# Autodesk Inventor assembly: mill_assembly
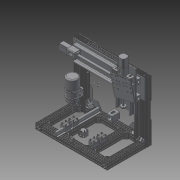
[picture p0: Inventor's stored thumbnail of the model, 180x180]
Saved by Autodesk Inventor 2014 (Build 180170000, 170)
## iProperties
Created: 2014-08-08
Part Number: mill_assembly
Document SubType Name: Assembly
Designer: Matthew
Author: Matthew
## Documents named in this file (43)
- C:\Users\matmell\Documents\GitHub\cncmill\mill_assembly.iam
- C:\Users\matmell\Documents\GitHub\cncmill\8020\2020.ipt
- C:\Users\matmell\Documents\GitHub\cncmill\8020\2020_18in.ipt
- C:\Users\matmell\Documents\GitHub\cncmill\8020\gusset_4138.ipt
- C:\Users\matmell\Documents\GitHub\cncmill\8020\gusset_4134.ipt
- C:\Users\matmell\Documents\GitHub\cncmill\mic6_plate.ipt
- C:\Users\matmell\Documents\GitHub\cncmill\1605\1605_400mm.ipt
- C:\Users\matmell\Documents\GitHub\cncmill\1605\1605_ballnut.ipt
- C:\Users\matmell\Documents\GitHub\cncmill\nema23_motor_mount.ipt
- C:\Users\matmell\Documents\GitHub\cncmill\6.35x10mm_coupler.ipt
- C:\Users\matmell\Documents\GitHub\cncmill\sbr\sbr20\sbr20_400mm.ipt
- C:\Users\matmell\Documents\GitHub\cncmill\HD16.ipt
- C:\Users\matmell\Documents\GitHub\cncmill\nema23_HS8630.ipt
- C:\Users\matmell\Documents\GitHub\cncmill\z-axis_mount_plate.ipt
- C:\Users\matmell\Documents\GitHub\cncmill\y-axis_mount_plate.ipt
- C:\Users\matmell\Documents\GitHub\cncmill\router_plate.ipt
- C:\Users\matmell\Documents\GitHub\cncmill\router_mount.ipt
- C:\Users\matmell\Documents\GitHub\cncmill\1617evs.ipt
- C:\Users\matmell\Documents\GitHub\cncmill\ff12_mount.ipt
- C:\Users\matmell\Documents\GitHub\cncmill\ff12.ipt
- C:\Users\matmell\Documents\GitHub\cncmill\sbr\sbr20\sbr20_500mm.ipt
- C:\Users\matmell\Documents\GitHub\cncmill\1605\1605_500mm.ipt
- C:\Users\matmell\Documents\GitHub\cncmill\sbr\sbr20\sbr20_300mm.ipt
- C:\Users\matmell\Documents\GitHub\cncmill\8020\2040_top_bar.ipt
- C:\Users\matmell\Documents\GitHub\cncmill\8020\2040_uprights.ipt
- C:\Users\matmell\Documents\GitHub\cncmill\8020\2020_rear.ipt
- C:\Users\matmell\Documents\GitHub\cncmill\8020\2020_front.ipt
- C:\Users\matmell\Documents\GitHub\cncmill\1605\1605_300mm.ipt
- C:\Users\matmell\Documents\GitHub\cncmill\versaframe\versaframe_30in.ipt
- C:\Users\matmell\Documents\GitHub\cncmill\versaframe\versaframe_35in.ipt
- C:\Users\matmell\Documents\GitHub\cncmill\versaframe\versaframe_7.5n.ipt
- C:\Users\matmell\Documents\GitHub\cncmill\8020\2040-2040_left.iam
- C:\Users\matmell\Documents\GitHub\cncmill\8020\2040-2040_right.iam
- C:\Users\matmell\Documents\GitHub\cncmill\8020\2020-2040_right.iam
- C:\Users\matmell\Documents\GitHub\cncmill\8020\2020-2040_left.iam
- C:\Users\matmell\Documents\GitHub\cncmill\fk12.ipt
- C:\Users\matmell\Documents\GitHub\cncmill\sbr\sbr20\sbr20uu.ipt
- C:\Users\matmell\Documents\GitHub\cncmill\m6x1.ipt
- C:\Users\matmell\Documents\GitHub\cncmill\m5x0.8.ipt
- C:\Users\matmell\Documents\GitHub\cncmill\8020\SHCS bolt.ipt
- C:\Users\matmell\Documents\GitHub\cncmill\8020\0.5in_tnut.iam
- C:\Users\matmell\Documents\GitHub\cncmill\Metric socket button head, Class 12.9 steel black oil finish, 5mm x.ipt
- C:\Users\matmell\Documents\GitHub\cncmill\Metric socket button head, Class 12.9 steel black oil finish, 6mm x 1.ipt
## Components (124 placed, 42 different names)
1. 2020_18in:1 — Mate:31, Mate:32, Mate:38, Mate:47, Mate:48, Flush:161, Flush:168, Mate:253
2. 2020_18in:2 — Mate:28, Mate:29, Mate:34, Mate:241, Flush:163, Mate:242, Flush:164, Mate:255, Flush:171, Flush:172, Mate:394
3. gusset_4138:1 — Mate:260, Mate:261, Flush:175
4. gusset_4138:2 — Mate:258, Mate:259, Mate:262, Flush:175
5. gusset_4134:1 — Mate:28, Mate:29, Mate:275
6. gusset_4134:2 — Mate:31, Mate:32, Mate:276, Insert:58, Insert:60, Insert:61, Insert:62
7. gusset_4134:3 — Mate:34, Flush:61, Flush:147, Mate:278
8. gusset_4134:4 — Mate:38, Flush:62, Flush:153, Mate:279
9. gusset_4134:6 — Mate:47, Mate:48, Flush:61, Flush:62, Mate:269, Flush:401, Flush:402, Flush:403
10. mic6_plate:1 — Insert:17, Insert:18, Insert:19, Insert:20, Insert:21, Insert:22, Insert:23, Insert:24, Insert:25, Insert:26, Insert:27, Insert:28, Insert:29, Insert:30, Insert:31, Insert:32, Insert:33, Insert:34, Insert:35, Insert:36, Flush:395, Mate:397
11. 1605_400mm:1 — Mate:108, Insert:2, Insert:16, Mate:404, Flush:408
12. 1605_ballnut:1 — Mate:108, Mate:133, Mate:134, Mate:408
13. nema23_motor_mount:1 — Mate:136, Mate:254, Flush:192, Flush:193, Mate:317, Flush:329, Flush:330, Flush:407
14. nema23_motor_mount:2 — Mate:154, Flush:321, Flush:322, Mate:316, Flush:327, Flush:328, Mate:364, Flush:376
15. 1605_ballnut:6 — Mate:158, Mate:159, Mate:282
16. 6.35x10mm_coupler:1 — Insert:4, Insert:14
17. sbr20_400mm:1 — Flush:136, Mate:247, Flush:191, Mate:318
18. sbr20_400mm:2 — Flush:136, Mate:248, Flush:190, Mate:328
19. HD16:1 — Mate:133, Mate:134, Mate:326, Mate:329, Mate:395, Mate:408
20. nema23_HS8630:1 — Mate:136, Flush:192, Flush:193
21. 6.35x10mm_coupler:2 — Insert:2
22. z-axis_mount_plate:1 — Flush:370, Flush:371, Flush:372, Flush:373, Mate:362, Mate:363, Flush:375, Mate:364, Flush:376, Flush:390, Mate:400, Angle:2
23. nema23_HS8630:2 — Mate:154, Insert:4, Flush:321, Flush:322
24. HD16:6 — Mate:158, Mate:159, Mate:210, Mate:211, Flush:390, Mate:405, Mate:406
25. y-axis_mount_plate:1 — Mate:177, Mate:199, Mate:200, Flush:135, Mate:206, Flush:137, Flush:184, Mate:267, Flush:396
26. nema23_motor_mount:4 — Mate:177, Flush:137, Flush:323, Flush:324, Mate:315, Flush:325, Flush:326
27. 6.35x10mm_coupler:3
28. nema23_HS8630:3 — Flush:323, Flush:324
29. 1605_ballnut:7 — Mate:240
30. HD16:7 — Mate:203, Mate:205, Mate:348
31. router_mount:1 — Insert:7
32. 1617evs:1 — Insert:7
33. ff12:1 — Mate:404, Flush:408, Angle:1
34. sbr20_500mm:1 — Flush:133, Mate:200, Mate:203, Flush:135, Mate:346, Flush:371, Mate:382
35. sbr20_500mm:2 — Flush:133, Mate:199, Mate:205, Mate:347
36. 1605_500mm:1 — Insert:11, Mate:240, Insert:15
37. ff12:2 — Insert:11, Insert:12
38. ff12_mount:2 — Insert:12, Mate:206
39. sbr20_300mm:1 — Flush:138, Mate:210, Flush:372, Mate:363, Flush:374, Flush:375, Mate:371
40. sbr20_300mm:2 — Flush:138, Mate:211, Flush:373, Mate:362, Flush:374, Mate:377
41. 2020:1 — Mate:223, Mate:230, Mate:233, Mate:248, Flush:169, Flush:190, Mate:389, Mate:398
42. 2020:2 — Mate:222, Mate:224, Mate:226, Mate:247, Flush:170, Flush:191, Mate:391, Mate:403
43. gusset_4134:8 — Mate:222, Flush:147, Mate:277
44. gusset_4134:9 — Mate:223, Flush:149, Flush:150, Flush:151, Mate:280, Flush:401
45. gusset_4134:11 — Mate:224, Flush:149, Mate:268
46. gusset_4134:12 — Mate:230, Flush:151, Mate:390
47. gusset_4134:13 — Mate:226, Flush:150, Mate:281
48. gusset_4134:14 — Flush:153, Mate:233
49. 2040_top_bar:1 — Mate:257, Flush:173, Flush:174, Mate:258, Mate:261, Flush:184, Mate:267, Flush:313, Flush:315
50. 2040_uprights:1 — Flush:161, Mate:241, Flush:167, Mate:252, Flush:168, Mate:253, Mate:257, Flush:173, Flush:174, Mate:259, Mate:262, Mate:269, Mate:276, Mate:311, Flush:314, Mate:314, Flush:319, Flush:320, Flush:396, Flush:398, Mate:385, Flush:400, Mate:395
51. 2040_uprights:2 — Flush:163, Mate:242, Flush:164, Mate:249, Flush:165, Flush:166, Mate:260, Mate:275, Flush:208, Mate:312, Flush:316, Mate:313, Flush:317, Flush:318, Mate:386, Flush:399, Flush:404, Mate:393
52. 2020_rear:1 — Mate:249, Flush:165, Flush:166, Flush:167, Mate:252, Flush:169, Flush:170, Mate:254, Mate:268, Mate:280, Flush:221, Mate:384, Mate:387, Mate:388, Mate:392, Flush:407
53. 2020_front:1 — Mate:255, Flush:171, Flush:172, Mate:277, Mate:278, Mate:279, Mate:281, Mate:390, Mate:398, Mate:403, Angle:1
54. 1605_300mm:1 — Insert:14, Mate:282, Insert:69
55. versaframe_30in:1 — Flush:200, Flush:201, Mate:294, Flush:202, Flush:203, Mate:295, Flush:205, Flush:206, Flush:228, Flush:230
56. versaframe_30in:2 — Flush:200, Flush:201, Flush:204, Flush:221
57. versaframe_35in:1 — Mate:294, Flush:202, Flush:203, Flush:204, Flush:208, Flush:213, Mate:303, Flush:229
58. versaframe_35in:2 — Mate:295, Flush:205, Flush:206, Mate:297, Flush:209, Flush:210, Mate:304, Flush:231
59. versaframe_30in:3 — Mate:297, Flush:209, Flush:210, Flush:211, Flush:212, Flush:232, Flush:233, Mate:305
60. versaframe_30in:4 — Flush:211, Flush:212, Flush:213, Flush:220, Flush:308, Flush:235, Flush:309
61. versaframe_7.5n:1 — Flush:308, Flush:235, Flush:309, Flush:310, Flush:311, Mate:307, Mate:308
62. versaframe_7.5n:2 — Flush:232, Flush:233, Mate:305, Mate:306, Flush:234, Mate:309, Mate:310, Flush:312
63. versaframe_30in:5 — Flush:220, Flush:222, Mate:306, Flush:234, Flush:310
64. versaframe_30in:6 — Flush:222, Flush:311, Mate:307, Mate:308
65. versaframe_7.5n:3 — Mate:303, Flush:228, Flush:229
66. versaframe_7.5n:4 — Mate:304, Flush:230, Flush:231
67. versaframe_30in:7
68. versaframe_30in:8 — Mate:309, Mate:310, Flush:312
69. 2040-2040_left:1 [sub-assembly] — Mate:311, Flush:313, Flush:314
70. 2040-2040_right:1 [sub-assembly] — Mate:312, Flush:315, Flush:316
71. 2020-2040_right:1 [sub-assembly] — Mate:313, Flush:317, Flush:318
72. 2020-2040_left:1 [sub-assembly] — Mate:314, Flush:319, Flush:320
73. fk12:1 — Insert:15, Mate:315, Flush:325, Flush:326, Mate:382
74. fk12:2 — Mate:316, Flush:327, Flush:328
75. fk12:3 — Mate:317, Flush:329, Flush:330, Insert:16
76. sbr20uu:1 — Flush:332, Mate:319, Flush:333, Mate:396, Mate:397
77. sbr20uu:2 — Mate:318, Flush:332, Mate:319, Flush:333, Mate:326, Flush:395, Flush:406
78. sbr20uu:3 — Flush:344, Mate:327, Flush:345, Mate:328, Mate:329, Flush:406
79. sbr20uu:13 — Flush:344, Mate:327, Flush:345
80. m6x1:1 — Insert:24
81. m6x1:2 — Insert:21
82. m6x1:3 — Insert:17
83. m6x1:4 — Insert:20
84. m6x1:5 — Insert:18
85. m6x1:6 — Insert:19
86. m6x1:7 — Insert:22
87. m6x1:8 — Insert:23
88. m6x1:9 — Insert:28
89. m6x1:10 — Insert:27
90. m6x1:11 — Insert:32, Mate:396
91. m6x1:12 — Insert:26
92. m6x1:13 — Insert:29
93. m6x1:14 — Insert:30
94. m6x1:15 — Insert:25
95. m6x1:16 — Insert:31
96. m5x0.8:1 — Insert:36
97. m5x0.8:2 — Insert:34
98. m5x0.8:3 — Insert:33
99. m5x0.8:4 — Insert:35
100. sbr20uu:14 — Mate:347, Flush:362, Mate:348, Flush:370
101. sbr20uu:15
102. sbr20uu:18 — Mate:346, Flush:362
103. sbr20uu:19 — Mate:400
104. sbr20uu:22 — Mate:371
105. sbr20uu:23 — Flush:387, Mate:407
106. sbr20uu:24
107. sbr20uu:25 — Mate:377, Flush:387
108. gusset_4138:5 — Mate:384, Flush:398, Mate:385
109. gusset_4138:6 — Mate:386, Flush:399, Mate:387
110. gusset_4134:15 — Mate:388, Mate:389, Flush:400, Flush:402
111. gusset_4134:16 — Mate:391, Flush:403, Flush:404, Mate:392, Flush:405
112. gusset_4134:17 — Mate:393, Mate:394, Flush:405
113. SHCS bolt:2 — Insert:58
114. 0.5in_tnut:2 [sub-assembly] — Insert:60
115. 0.5in_tnut:3 [sub-assembly] — Insert:61
116. SHCS bolt:3 — Insert:62
117. Metric socket button head, Class 12.9 steel black oil finish, 5mm x:1
118. Metric socket button head, Class 12.9 steel black oil finish, 5mm x:2 — Mate:405
119. Metric socket button head, Class 12.9 steel black oil finish, 5mm x:3
120. Metric socket button head, Class 12.9 steel black oil finish, 5mm x:4
121. Metric socket button head, Class 12.9 steel black oil finish, 6mm x 1:1
122. Metric socket button head, Class 12.9 steel black oil finish, 6mm x 1:2
123. ff12:3 — Insert:69, Angle:2
124. router_plate:1 — Mate:406, Mate:407
## Relationships (267: Mate 118, Flush 113, Insert 34, Angle 2)
- Mate:28: 2020_18in:2 ↔ gusset_4134:1
- Mate:29: 2020_18in:2 ↔ gusset_4134:1
- Mate:31: 2020_18in:1 ↔ gusset_4134:2
- Mate:32: 2020_18in:1 ↔ gusset_4134:2
- Mate:34: 2020_18in:2 ↔ gusset_4134:3
- Mate:38: 2020_18in:1 ↔ gusset_4134:4
- Mate:47: 2020_18in:1 ↔ gusset_4134:6
- Mate:48: 2020_18in:1 ↔ gusset_4134:6
- Mate:108: 1605_400mm:1 ↔ 1605_ballnut:1
- Flush:61: gusset_4134:3 ↔ gusset_4134:6
- Flush:62: gusset_4134:4 ↔ gusset_4134:6
- Mate:133: 1605_ballnut:1 ↔ HD16:1
- Mate:134: 1605_ballnut:1 ↔ HD16:1
- Insert:2 (-12.5 mm): 1605_400mm:1 ↔ 6.35x10mm_coupler:2
- Mate:136: nema23_motor_mount:1 ↔ nema23_HS8630:1
- Mate:154: nema23_motor_mount:2 ↔ nema23_HS8630:2
- Insert:4 (-7 mm): 6.35x10mm_coupler:1 ↔ nema23_HS8630:2
- Mate:158: 1605_ballnut:6 ↔ HD16:6
- Mate:159: 1605_ballnut:6 ↔ HD16:6
- [Mate]: nema23_motor_mount:4 ↔ nema23_HS8630:3
- [Insert] (-7 mm): 6.35x10mm_coupler:3 ↔ nema23_HS8630:3
- [Mate]: 1605_ballnut:7 ↔ HD16:7
- [Mate]: 1605_ballnut:7 ↔ HD16:7
- Mate:177: y-axis_mount_plate:1 ↔ nema23_motor_mount:4
- Insert:7: router_mount:1 ↔ 1617evs:1
- Flush:133: sbr20_500mm:1 ↔ sbr20_500mm:2
- Mate:199: y-axis_mount_plate:1 ↔ sbr20_500mm:2
- Mate:200: y-axis_mount_plate:1 ↔ sbr20_500mm:1
- Mate:203 (19.9 mm): HD16:7 ↔ sbr20_500mm:1
- Mate:205 (19.9 mm): HD16:7 ↔ sbr20_500mm:2
- Flush:135: y-axis_mount_plate:1 ↔ sbr20_500mm:1
- Flush:136: sbr20_400mm:1 ↔ sbr20_400mm:2
- Insert:11: 1605_500mm:1 ↔ ff12:2
- Insert:12: ff12:2 ↔ ff12_mount:2
- Mate:206: y-axis_mount_plate:1 ↔ ff12_mount:2
- Flush:137: y-axis_mount_plate:1 ↔ nema23_motor_mount:4
- Flush:138: sbr20_300mm:1 ↔ sbr20_300mm:2
- Mate:210 (11 mm): HD16:6 ↔ sbr20_300mm:1
- Mate:211 (11 mm): HD16:6 ↔ sbr20_300mm:2
- Mate:222: 2020:2 ↔ gusset_4134:8
- Flush:147: gusset_4134:3 ↔ gusset_4134:8
- Mate:223: 2020:1 ↔ gusset_4134:9
- Mate:224: 2020:2 ↔ gusset_4134:11
- Mate:226: 2020:2 ↔ gusset_4134:13
- Flush:149: gusset_4134:9 ↔ gusset_4134:11
- Mate:230: 2020:1 ↔ gusset_4134:12
- Flush:150: gusset_4134:9 ↔ gusset_4134:13
- Flush:151: gusset_4134:9 ↔ gusset_4134:12
- Flush:153: gusset_4134:4 ↔ gusset_4134:14
- Mate:233: 2020:1 ↔ gusset_4134:14
- Mate:240: 1605_ballnut:7 ↔ 1605_500mm:1
- Flush:161: 2020_18in:1 ↔ 2040_uprights:1
- Mate:241: 2020_18in:2 ↔ 2040_uprights:1
- Flush:163: 2020_18in:2 ↔ 2040_uprights:2
- Mate:242: 2020_18in:2 ↔ 2040_uprights:2
- Flush:164: 2020_18in:2 ↔ 2040_uprights:2
- Mate:247: sbr20_400mm:1 ↔ 2020:2
- Mate:248: sbr20_400mm:2 ↔ 2020:1
- Mate:249: 2040_uprights:2 ↔ 2020_rear:1
- Flush:165: 2040_uprights:2 ↔ 2020_rear:1
- Flush:166: 2040_uprights:2 ↔ 2020_rear:1
- Flush:167: 2040_uprights:1 ↔ 2020_rear:1
- Mate:252: 2040_uprights:1 ↔ 2020_rear:1
- Flush:168: 2020_18in:1 ↔ 2040_uprights:1
- Mate:253: 2020_18in:1 ↔ 2040_uprights:1
- Flush:169: 2020:1 ↔ 2020_rear:1
- Flush:170: 2020:2 ↔ 2020_rear:1
- Mate:254: nema23_motor_mount:1 ↔ 2020_rear:1
- Mate:255: 2020_18in:2 ↔ 2020_front:1
- Flush:171: 2020_18in:2 ↔ 2020_front:1
- Flush:172: 2020_18in:2 ↔ 2020_front:1
- Mate:257: 2040_top_bar:1 ↔ 2040_uprights:1
- Flush:173: 2040_top_bar:1 ↔ 2040_uprights:1
- Flush:174: 2040_top_bar:1 ↔ 2040_uprights:1
- Mate:258: gusset_4138:2 ↔ 2040_top_bar:1
- Mate:259: gusset_4138:2 ↔ 2040_uprights:1
- Mate:260: gusset_4138:1 ↔ 2040_uprights:2
- Mate:261: gusset_4138:1 ↔ 2040_top_bar:1
- Mate:262: gusset_4138:2 ↔ 2040_uprights:1
- Flush:175: gusset_4138:1 ↔ gusset_4138:2
- Flush:184: y-axis_mount_plate:1 ↔ 2040_top_bar:1
- Mate:267: y-axis_mount_plate:1 ↔ 2040_top_bar:1
- Mate:268: gusset_4134:11 ↔ 2020_rear:1
- Mate:269: gusset_4134:6 ↔ 2040_uprights:1
- Flush:190: sbr20_400mm:2 ↔ 2020:1
- Flush:191: sbr20_400mm:1 ↔ 2020:2
- Mate:275: gusset_4134:1 ↔ 2040_uprights:2
- Mate:276: gusset_4134:2 ↔ 2040_uprights:1
- Mate:277: gusset_4134:8 ↔ 2020_front:1
- Mate:278: gusset_4134:3 ↔ 2020_front:1
- Mate:279: gusset_4134:4 ↔ 2020_front:1
- Mate:280: gusset_4134:9 ↔ 2020_rear:1
- Mate:281: gusset_4134:13 ↔ 2020_front:1
- Insert:14 (-12.5 mm): 6.35x10mm_coupler:1 ↔ 1605_300mm:1
- Mate:282: 1605_ballnut:6 ↔ 1605_300mm:1
- Flush:192 (-0.889 mm): nema23_motor_mount:1 ↔ nema23_HS8630:1
- Flush:193: nema23_motor_mount:1 ↔ nema23_HS8630:1
- Flush:200: versaframe_30in:1 ↔ versaframe_30in:2
- Flush:201: versaframe_30in:1 ↔ versaframe_30in:2
- Mate:294: versaframe_30in:1 ↔ versaframe_35in:1
- Flush:202: versaframe_30in:1 ↔ versaframe_35in:1
- Flush:203: versaframe_30in:1 ↔ versaframe_35in:1
- Flush:204: versaframe_30in:2 ↔ versaframe_35in:1
- Mate:295: versaframe_30in:1 ↔ versaframe_35in:2
- Flush:205: versaframe_30in:1 ↔ versaframe_35in:2
- Flush:206: versaframe_30in:1 ↔ versaframe_35in:2
- Flush:208: 2040_uprights:2 ↔ versaframe_35in:1
- Mate:297: versaframe_35in:2 ↔ versaframe_30in:3
- Flush:209: versaframe_35in:2 ↔ versaframe_30in:3
- Flush:210: versaframe_35in:2 ↔ versaframe_30in:3
- Flush:211: versaframe_30in:3 ↔ versaframe_30in:4
- Flush:212: versaframe_30in:3 ↔ versaframe_30in:4
- Flush:213: versaframe_35in:1 ↔ versaframe_30in:4
- Flush:220: versaframe_30in:4 ↔ versaframe_30in:5
- Flush:221: 2020_rear:1 ↔ versaframe_30in:2
- Flush:222: versaframe_30in:5 ↔ versaframe_30in:6
- Mate:303: versaframe_35in:1 ↔ versaframe_7.5n:3
- Flush:228: versaframe_30in:1 ↔ versaframe_7.5n:3
- Flush:229: versaframe_35in:1 ↔ versaframe_7.5n:3
- Mate:304: versaframe_35in:2 ↔ versaframe_7.5n:4
- Flush:230: versaframe_30in:1 ↔ versaframe_7.5n:4
- Flush:231: versaframe_35in:2 ↔ versaframe_7.5n:4
- Flush:232: versaframe_30in:3 ↔ versaframe_7.5n:2
- Flush:233: versaframe_30in:3 ↔ versaframe_7.5n:2
- Mate:305: versaframe_30in:3 ↔ versaframe_7.5n:2
- Mate:306: versaframe_7.5n:2 ↔ versaframe_30in:5
- Flush:234: versaframe_7.5n:2 ↔ versaframe_30in:5
- Flush:308: versaframe_30in:4 ↔ versaframe_7.5n:1
- Flush:235: versaframe_30in:4 ↔ versaframe_7.5n:1
- Flush:309: versaframe_30in:4 ↔ versaframe_7.5n:1
- Flush:310: versaframe_7.5n:1 ↔ versaframe_30in:5
- Flush:311: versaframe_7.5n:1 ↔ versaframe_30in:6
- Mate:307: versaframe_7.5n:1 ↔ versaframe_30in:6
- Mate:308: versaframe_7.5n:1 ↔ versaframe_30in:6
- Mate:309: versaframe_7.5n:2 ↔ versaframe_30in:8
- Mate:310: versaframe_7.5n:2 ↔ versaframe_30in:8
- Flush:312: versaframe_7.5n:2 ↔ versaframe_30in:8
- Mate:311: 2040_uprights:1 ↔ 2040-2040_left:1
- Flush:313: 2040_top_bar:1 ↔ 2040-2040_left:1
- Flush:314: 2040_uprights:1 ↔ 2040-2040_left:1
- Mate:312: 2040_uprights:2 ↔ 2040-2040_right:1
- Flush:315: 2040_top_bar:1 ↔ 2040-2040_right:1
- Flush:316: 2040_uprights:2 ↔ 2040-2040_right:1
- Mate:313: 2040_uprights:2 ↔ 2020-2040_right:1
- Flush:317: 2040_uprights:2 ↔ 2020-2040_right:1
- Flush:318: 2040_uprights:2 ↔ 2020-2040_right:1
- Mate:314: 2040_uprights:1 ↔ 2020-2040_left:1
- Flush:319: 2040_uprights:1 ↔ 2020-2040_left:1
- Flush:320: 2040_uprights:1 ↔ 2020-2040_left:1
- Flush:321 (-0.889 mm): nema23_motor_mount:2 ↔ nema23_HS8630:2
- Flush:322 (0.889 mm): nema23_motor_mount:2 ↔ nema23_HS8630:2
- Flush:323 (-0.889 mm): nema23_motor_mount:4 ↔ nema23_HS8630:3
- Flush:324: nema23_motor_mount:4 ↔ nema23_HS8630:3
- Insert:15: 1605_500mm:1 ↔ fk12:1
- Mate:315: nema23_motor_mount:4 ↔ fk12:1
- Flush:325 (6.1305 mm): nema23_motor_mount:4 ↔ fk12:1
- Flush:326 (6.1305 mm): nema23_motor_mount:4 ↔ fk12:1
- Mate:316: nema23_motor_mount:2 ↔ fk12:2
- Flush:327 (-6.1305 mm): nema23_motor_mount:2 ↔ fk12:2
- Flush:328 (6.1305 mm): nema23_motor_mount:2 ↔ fk12:2
- Mate:317: nema23_motor_mount:1 ↔ fk12:3
- Flush:329 (6.1305 mm): nema23_motor_mount:1 ↔ fk12:3
- Flush:330 (6.1305 mm): nema23_motor_mount:1 ↔ fk12:3
- Insert:16: 1605_400mm:1 ↔ fk12:3
- Mate:318: sbr20_400mm:1 ↔ sbr20uu:2
- Flush:332: sbr20uu:1 ↔ sbr20uu:2
- Mate:319 (20 mm): sbr20uu:1 ↔ sbr20uu:2
- Flush:333: sbr20uu:1 ↔ sbr20uu:2
- Mate:326 (-7.5 mm): HD16:1 ↔ sbr20uu:2
- Flush:344: sbr20uu:3 ↔ sbr20uu:13
- Mate:327 (20 mm): sbr20uu:3 ↔ sbr20uu:13
- Flush:345: sbr20uu:3 ↔ sbr20uu:13
- Mate:328: sbr20_400mm:2 ↔ sbr20uu:3
- Mate:329 (-7.5 mm): HD16:1 ↔ sbr20uu:3
- Insert:17: mic6_plate:1 ↔ m6x1:3
- Insert:18: mic6_plate:1 ↔ m6x1:5
- Insert:19: mic6_plate:1 ↔ m6x1:6
- Insert:20: mic6_plate:1 ↔ m6x1:4
- Insert:21: mic6_plate:1 ↔ m6x1:2
- Insert:22: mic6_plate:1 ↔ m6x1:7
- Insert:23: mic6_plate:1 ↔ m6x1:8
- Insert:24: mic6_plate:1 ↔ m6x1:1
- Insert:25: mic6_plate:1 ↔ m6x1:15
- Insert:26: mic6_plate:1 ↔ m6x1:12
- Insert:27: mic6_plate:1 ↔ m6x1:10
- Insert:28: mic6_plate:1 ↔ m6x1:9
- Insert:29: mic6_plate:1 ↔ m6x1:13
- Insert:30: mic6_plate:1 ↔ m6x1:14
- Insert:31: mic6_plate:1 ↔ m6x1:16
- Insert:32: mic6_plate:1 ↔ m6x1:11
- Insert:33: mic6_plate:1 ↔ m5x0.8:3
- Insert:34: mic6_plate:1 ↔ m5x0.8:2
- Insert:35: mic6_plate:1 ↔ m5x0.8:4
- Insert:36: mic6_plate:1 ↔ m5x0.8:1
- [Flush]: sbr20uu:14 ↔ sbr20uu:15
- [Mate] (60 mm): sbr20uu:14 ↔ sbr20uu:15
- [Flush]: sbr20uu:14 ↔ sbr20uu:15
- [Flush]: sbr20uu:18 ↔ sbr20uu:19
- [Mate] (70 mm): sbr20uu:18 ↔ sbr20uu:19
- [Flush]: sbr20uu:18 ↔ sbr20uu:19
- Mate:346: sbr20_500mm:1 ↔ sbr20uu:18
- Mate:347: sbr20_500mm:2 ↔ sbr20uu:14
- Flush:362: sbr20uu:14 ↔ sbr20uu:18
- Mate:348 (12.5 mm): HD16:7 ↔ sbr20uu:14
- Flush:370: z-axis_mount_plate:1 ↔ sbr20uu:14
- Flush:371 (-91.0209 mm): z-axis_mount_plate:1 ↔ sbr20_500mm:1
- Flush:372: z-axis_mount_plate:1 ↔ sbr20_300mm:1
- Flush:373: z-axis_mount_plate:1 ↔ sbr20_300mm:2
- Mate:362: z-axis_mount_plate:1 ↔ sbr20_300mm:2
- Mate:363: z-axis_mount_plate:1 ↔ sbr20_300mm:1
- Flush:374: sbr20_300mm:1 ↔ sbr20_300mm:2
- Flush:375: z-axis_mount_plate:1 ↔ sbr20_300mm:1
- Mate:364: nema23_motor_mount:2 ↔ z-axis_mount_plate:1
- Flush:376: nema23_motor_mount:2 ↔ z-axis_mount_plate:1
- [Flush]: sbr20uu:22 ↔ sbr20uu:23
- [Mate] (10 mm): sbr20uu:22 ↔ sbr20uu:23
- [Flush]: sbr20uu:22 ↔ sbr20uu:23
- Mate:371: sbr20_300mm:1 ↔ sbr20uu:22
- [Flush]: sbr20uu:24 ↔ sbr20uu:25
- [Mate] (10 mm): sbr20uu:24 ↔ sbr20uu:25
- [Flush]: sbr20uu:24 ↔ sbr20uu:25
- Mate:377: sbr20_300mm:2 ↔ sbr20uu:25
- Flush:387: sbr20uu:23 ↔ sbr20uu:25
- Flush:390 (61 mm): z-axis_mount_plate:1 ↔ HD16:6
- Mate:382 (-40 mm): sbr20_500mm:1 ↔ fk12:1
- Flush:395 (-92.4 mm): mic6_plate:1 ↔ sbr20uu:2
- Flush:396: y-axis_mount_plate:1 ↔ 2040_uprights:1
- Mate:384: 2020_rear:1 ↔ gusset_4138:5
- Flush:398: 2040_uprights:1 ↔ gusset_4138:5
- Mate:385: 2040_uprights:1 ↔ gusset_4138:5
- Mate:386: 2040_uprights:2 ↔ gusset_4138:6
- Flush:399: 2040_uprights:2 ↔ gusset_4138:6
- Mate:387: 2020_rear:1 ↔ gusset_4138:6
- Mate:388: 2020_rear:1 ↔ gusset_4134:15
- Mate:389: 2020:1 ↔ gusset_4134:15
- Flush:400 (-76.2 mm): 2040_uprights:1 ↔ gusset_4134:15
- Mate:390: gusset_4134:12 ↔ 2020_front:1
- Flush:401: gusset_4134:6 ↔ gusset_4134:9
- Flush:402: gusset_4134:6 ↔ gusset_4134:15
- Mate:391: 2020:2 ↔ gusset_4134:16
- Flush:403: gusset_4134:6 ↔ gusset_4134:16
- Flush:404 (-76.2 mm): 2040_uprights:2 ↔ gusset_4134:16
- Mate:392: 2020_rear:1 ↔ gusset_4134:16
- Mate:393: 2040_uprights:2 ↔ gusset_4134:17
- Mate:394: 2020_18in:2 ↔ gusset_4134:17
- Flush:405: gusset_4134:16 ↔ gusset_4134:17
- Insert:58: gusset_4134:2 ↔ SHCS bolt:2
- Insert:60: gusset_4134:2 ↔ 0.5in_tnut:2
- Insert:61: gusset_4134:2 ↔ 0.5in_tnut:3
- Insert:62: gusset_4134:2 ↔ SHCS bolt:3
- Flush:406: sbr20uu:2 ↔ sbr20uu:3
- Mate:395 (204.6 mm): HD16:1 ↔ 2040_uprights:1
- Mate:396: sbr20uu:1 ↔ m6x1:11
- Mate:397: mic6_plate:1 ↔ sbr20uu:1
- Mate:398: 2020:1 ↔ 2020_front:1
- Mate:400: z-axis_mount_plate:1 ↔ sbr20uu:19
- Mate:403: 2020:2 ↔ 2020_front:1
- Flush:407 (-3.175 mm): nema23_motor_mount:1 ↔ 2020_rear:1
- Mate:404: 1605_400mm:1 ↔ ff12:1
- Flush:408 (2 mm): 1605_400mm:1 ↔ ff12:1
- Angle:1 (180 deg): ff12:1 ↔ 2020_front:1
- Insert:69: 1605_300mm:1 ↔ ff12:3
- Angle:2 (90.08 deg): z-axis_mount_plate:1 ↔ ff12:3
- Mate:405 (1.2192 mm): HD16:6 ↔ Metric socket button head, Class 12.9 steel black oil finish, 5mm x:2
- Mate:406: HD16:6 ↔ router_plate:1
- Mate:407: sbr20uu:23 ↔ router_plate:1
- Mate:408: 1605_ballnut:1 ↔ HD16:1
## Named parameters: d373_d340 = -7 mm, d376_d338 = 0 mm, d379_d346 = 0 mm, d381_d348 = 0 mm, yaxissbrspacing = 19.9 mm, zaxismount = 359.8418 mm, motoroffset = -0.889 mm, fk12offset = 6.1305 mm, d865_d806_d803_d800 = 0 mm, d866_d807_d804_d801 = 60 mm, d867_d808_d805_d802 = 0 mm, d876_d865_d806_d803_d800 = 0 mm, d877_d866_d807_d804_d801 = 70 mm, d878_d867_d808_d805_d802 = 0 mm, d919_d876_d865_d806_d803_d800 = 0 mm, d920_d877_d866_d807_d804_d801 = 10 mm, d921_d878_d867_d808_d805_d802 = 0 mm, d929_d919_d876_d865_d806_d803_d800 = 0 mm, d930_d920_d877_d866_d807_d804_d801 = 10 mm, d931_d921_d878_d867_d808_d805_d802 = 0 mm
